# Autodesk Inventor assembly: x_carryage
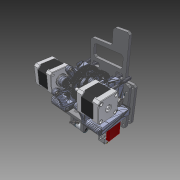
[picture p0: Inventor's stored thumbnail of the model, 180x180]
Saved by Autodesk Inventor 2014 (Build 180170000, 170)
## iProperties
Created: 2014-03-26
Part Number: x_carryage
Document SubType Name: Assembly
Designer: buben
Mass: 379.777 g
Surface Area: 1487.79 cm^2
Volume: 289.429 cm^3
Density: 1.31216 g/cm^3
Author: buben
## Documents named in this file (10)
- C:\Users\buben\Documents\GitHub\bacon\inventor files\printer parts\6.5 mm\x_carryage.iam
- C:\Users\buben\Documents\GitHub\bacon\inventor files\printer parts\6.5 mm\x_carryage_extruder_mount.ipt
- C:\Users\buben\Documents\GitHub\bacon\inventor files\assemblies\extruder.iam
- C:\Users\buben\Documents\GitHub\bacon\inventor files\printer parts\6.5 mm\x_carryage_front.ipt
- C:\Users\buben\Documents\GitHub\bacon\inventor files\3rd party components\linear_bearing_8\Imported Components\LU8MM\LU8MM.iam
- C:\Users\buben\Documents\GitHub\bacon\inventor files\utils\hotend_cooling_mount.ipt
- C:\Users\buben\Documents\GitHub\bacon\inventor files\assemblies\extruder_mirrored.iam
- C:\Users\buben\Documents\GitHub\bacon\inventor files\printer parts\6.5 mm\x_carryage_back.ipt
- C:\Users\buben\Documents\GitHub\bacon\inventor files\printer parts\6.5 mm\x_carryage_brace_bottom.ipt
- C:\Users\buben\Documents\GitHub\bacon\inventor files\printer parts\6.5 mm\x_carryage_brace_top.ipt
## Components (15 placed, 9 different names)
1. x_carryage_extruder_mount:1 — Mate:2, Mate:3, Flush:2, Mate:20, Angle:3, Mate:23, Mate:24, Mate:25, Angle:4, Mate:26, Mate:31, Mate:32, Mate:35, Mate:37, Mate:38, Mate:39
2. extruder:1 [sub-assembly] — Mate:2, Mate:17, Flush:3, Mate:20, Angle:3
3. x_carryage_front:1 — Mate:3, Flush:2, Mate:4, Mate:5, Mate:6, Mate:7, Mate:8, Mate:9, Mate:10, Mate:11, Mate:12, Mate:13, Mate:14, Mate:15, Mate:21, Mate:22, Mate:24, Flush:7, Mate:33, Mate:34, Mate:36, Angle:5, Angle:6
4. LU8MM:1 [sub-assembly] — Mate:6, Mate:7, Mate:15
5. LU8MM:2 [sub-assembly] — Mate:4, Mate:5, Mate:13, Mate:30
6. LU8MM:3 [sub-assembly] — Mate:10, Mate:11, Mate:14
7. LU8MM:4 [sub-assembly] — Mate:8, Mate:9, Mate:12, Mate:28, Mate:29
8. hotend_cooling_mount:1 — Mate:17, Flush:3, Angle:5
9. extruder_mirrored:1 [sub-assembly] — Mate:25, Angle:4, Mate:26, Mate:27, Flush:6
10. hotend_cooling_mount:2 — Mate:27, Flush:6, Angle:6
11. x_carryage_back:1 — Mate:28, Mate:29, Mate:30, Flush:7
12. x_carryage_brace_bottom:1 — Mate:31, Mate:33, Mate:37
13. x_carryage_brace_bottom:2 — Mate:32, Mate:34, Mate:38, Mate:40
14. x_carryage_brace_top:1 — Mate:35, Mate:36, Mate:39
15. LU8MM:5 [sub-assembly] — Mate:40
## Relationships (44: Mate 36, Flush 4, Angle 4)
- Mate:2: x_carryage_extruder_mount:1 ↔ extruder:1
- Mate:3: x_carryage_extruder_mount:1 ↔ x_carryage_front:1
- Flush:2: x_carryage_extruder_mount:1 ↔ x_carryage_front:1
- Mate:4 (7.5 mm): x_carryage_front:1 ↔ LU8MM:2
- Mate:5 (7.5 mm): x_carryage_front:1 ↔ LU8MM:2
- Mate:6 (7.5 mm): x_carryage_front:1 ↔ LU8MM:1
- Mate:7 (7.5 mm): x_carryage_front:1 ↔ LU8MM:1
- Mate:8 (7.5 mm): x_carryage_front:1 ↔ LU8MM:4
- Mate:9 (7.5 mm): x_carryage_front:1 ↔ LU8MM:4
- Mate:10 (7.5 mm): x_carryage_front:1 ↔ LU8MM:3
- Mate:11 (7.5 mm): x_carryage_front:1 ↔ LU8MM:3
- Mate:12 (0.5 mm): x_carryage_front:1 ↔ LU8MM:4
- Mate:13 (0.5 mm): x_carryage_front:1 ↔ LU8MM:2
- Mate:14 (0.5 mm): x_carryage_front:1 ↔ LU8MM:3
- Mate:15 (0.5 mm): x_carryage_front:1 ↔ LU8MM:1
- Mate:17: extruder:1 ↔ hotend_cooling_mount:1
- Flush:3: extruder:1 ↔ hotend_cooling_mount:1
- Mate:20: x_carryage_extruder_mount:1 ↔ extruder:1
- Angle:3 (0 deg): x_carryage_extruder_mount:1 ↔ extruder:1
- Mate:21: x_carryage_front:1
- Mate:22: x_carryage_front:1
- Mate:23: x_carryage_extruder_mount:1
- Mate:24: x_carryage_extruder_mount:1 ↔ x_carryage_front:1
- Mate:25: x_carryage_extruder_mount:1 ↔ extruder_mirrored:1
- Angle:4 (0 deg): x_carryage_extruder_mount:1 ↔ extruder_mirrored:1
- Mate:26: x_carryage_extruder_mount:1 ↔ extruder_mirrored:1
- Mate:27: extruder_mirrored:1 ↔ hotend_cooling_mount:2
- Flush:6: extruder_mirrored:1 ↔ hotend_cooling_mount:2
- Mate:28 (7.5 mm): LU8MM:4 ↔ x_carryage_back:1
- Mate:29 (7.5 mm): LU8MM:4 ↔ x_carryage_back:1
- Mate:30 (7.5 mm): LU8MM:2 ↔ x_carryage_back:1
- Flush:7: x_carryage_front:1 ↔ x_carryage_back:1
- Mate:31: x_carryage_extruder_mount:1 ↔ x_carryage_brace_bottom:1
- Mate:32: x_carryage_extruder_mount:1 ↔ x_carryage_brace_bottom:2
- Mate:33: x_carryage_front:1 ↔ x_carryage_brace_bottom:1
- Mate:34: x_carryage_front:1 ↔ x_carryage_brace_bottom:2
- Mate:35: x_carryage_extruder_mount:1 ↔ x_carryage_brace_top:1
- Mate:36: x_carryage_front:1 ↔ x_carryage_brace_top:1
- Mate:37: x_carryage_extruder_mount:1 ↔ x_carryage_brace_bottom:1
- Mate:38: x_carryage_extruder_mount:1 ↔ x_carryage_brace_bottom:2
- Mate:39: x_carryage_extruder_mount:1 ↔ x_carryage_brace_top:1
- Angle:5 (180 deg): x_carryage_front:1 ↔ hotend_cooling_mount:1
- Angle:6 (180 deg): x_carryage_front:1 ↔ hotend_cooling_mount:2
- Mate:40: x_carryage_brace_bottom:2 ↔ LU8MM:5
